# Autodesk Inventor assembly: full
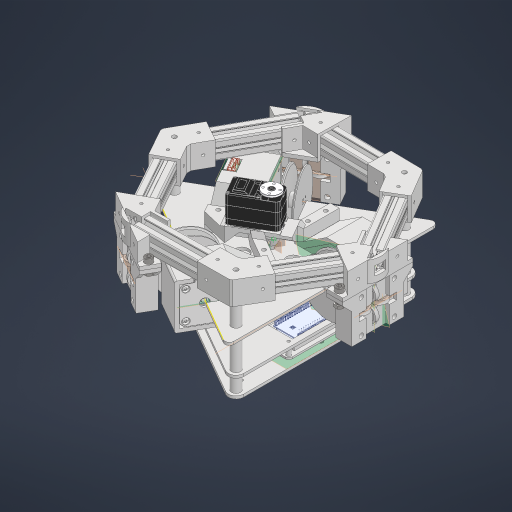
[picture p0: Inventor's stored thumbnail of the model, 512x512]
Saved by Autodesk Inventor 2024 (Build 280153000, 153)
## iProperties
Created: 2026-03-23
Part Number: full
Document SubType Name: Assembly
Designer: schar
Author: schar
## Documents named in this file (26)
- C:\Users\schar\Desktop\FloatingFace\models\full.iam
- C:\Users\schar\Desktop\FloatingFace\models\baseplate.ipt
- C:\Users\schar\Desktop\FloatingFace\models\spool.ipt
- C:\Users\schar\Desktop\FloatingFace\models\17HS4401S_Stepper_Motor\17HS4401S_Stepper_Motor.iam
- C:\Users\schar\Desktop\FloatingFace\models\esp32-s3-wroom-1-1.snapshot.2\ESP32-S3-WROOM-1\ESP32-S3-WROOM-1.iam
- C:\Users\schar\Desktop\FloatingFace\models\nema_brackets_and_lineguides.ipt
- C:\Users\schar\3D Objects\spacer_etage.ipt
- C:\Users\schar\3D Objects\second_etage.ipt
- C:\Users\schar\3D Objects\esp_spacer_fixed.ipt
- C:\Users\schar\Desktop\FloatingFace\models\esp_plate.ipt
- C:\Users\schar\Desktop\FloatingFace\models\guide.iam
- C:\Users\schar\Desktop\FloatingFace\models\2020_guide_adaptor.ipt
- C:\Users\schar\Desktop\FloatingFace\models\2020_top_guide_mnt.ipt
- C:\Users\schar\Desktop\FloatingFace\models\2020_nodes_conn.ipt
- C:\Users\schar\Desktop\FloatingFace\models\spacer_2020_node.ipt
- C:\Users\schar\Desktop\FloatingFace\models\2020_extrusion.ipt
- C:\Users\schar\Desktop\FloatingFace\models\ST3215 Servo.iam
- C:\Users\schar\Desktop\FloatingFace\models\servo_holder.ipt
- C:\Users\schar\Desktop\FloatingFace\models\servo_board_spacer.ipt
- C:\Users\schar\Desktop\FloatingFace\models\servo_rod_connector.ipt
- C:\Users\schar\Downloads\ROBOTIC_DOG_-STEP\drivers_pcb_v1.1.ipt
- C:\Users\schar\Desktop\FloatingFace\models\vertix_rod.ipt
- C:\Users\schar\Desktop\FloatingFace\models\multifunctional_lvl.ipt
- C:\Users\schar\Desktop\FloatingFace\models\multif_lvl_spacer.ipt
- C:\Users\schar\Documents\Inventor\Content Center Files\R2024\en-US\DIN 912\DIN 912 - M5 x 0,8 x 12 x 10.ipt
- C:\Users\schar\Documents\Inventor\Content Center Files\R2024\en-US\DIN 934\DIN 934 - M5 x 0,8.ipt
## Components (66 placed, 25 different names)
1. baseplate:1 — Mate:1, Mate:2, Mate:3, Mate:11, Mate:12, Flush:1, Mate:13, Mate:14, Mate:15, Flush:2, Flush:3, Flush:11, Flush:13, Mate:18, Mate:19, Mate:20, Mate:21, Flush:15, Mate:22, Mate:23, Angle:2, Angle:4, Flush:28, Mate:37, Mate:76, Mate:77, Mate:78
2. spool:1 — Mate:1, Mate:2, Mate:4, Mate:5
3. 17HS4401S_Stepper_Motor:1 [sub-assembly] — Mate:3, Mate:4, Mate:5
4. ESP32-S3-WROOM-1:1 [sub-assembly] — Mate:32, Flush:18, Flush:19
5. spool:2
6. 17HS4401S_Stepper_Motor:4 [sub-assembly] — Mate:14, Mate:15, Flush:2, Mate:16, Mate:17
7. spool:3 — Mate:11, Flush:4, Flush:20, Tangent:1, Tangent:2, Flush:24
8. 17HS4401S_Stepper_Motor:5 [sub-assembly] — Mate:12, Flush:1, Mate:13
9. nema_brackets_and_lineguides:1 — Flush:3, Flush:4, Flush:10, Angle:3, Angle:5
10. nema_brackets_and_lineguides:2 — Mate:16, Flush:11, Mate:17, Flush:12
11. spacer_etage:1 — Flush:13
12. spacer_etage:2 — Mate:18, Mate:19, Flush:14, Mate:31
13. spacer_etage:3 — Mate:20, Mate:21
14. second_etage:1 — Flush:14, Flush:16, Mate:25, Mate:26, Mate:27, Mate:28, Mate:29, Mate:30, Mate:31, Flush:35, Mate:80, Mate:81, Mate:82, Mate:83, Mate:84, Mate:85, Flush:41, Mate:86, Mate:87, Mate:88, Mate:89, Mate:90, Mate:91
15. nema_brackets_and_lineguides:3 — Flush:15, Mate:22, Mate:23, Mate:35, Flush:37
16. esp_spacer_fixed:1 — Flush:16, Flush:17
17. esp_spacer_fixed:2 — Mate:25, Mate:30
18. esp_spacer_fixed:3 — Mate:26, Mate:29
19. esp_spacer_fixed:4 — Mate:27, Mate:28
20. esp_plate:1 — Flush:17, Mate:32, Flush:18, Flush:19, Flush:39
21. drivers_pcb_v1.1:1
22. guide:2 [sub-assembly] — Mate:72, Mate:73, Mate:74
23. guide:3 [sub-assembly] — Mate:69, Mate:70, Mate:71
24. guide:1 [sub-assembly] — Mate:36, Flush:23, Flush:24, Flush:25
25. 2020_guide_adaptor:1 — Flush:25, Flush:26, Mate:104, Mate:106
26. 2020_top_guide_mnt:1 — Flush:26, Flush:29, Mate:55, Mate:56, Mate:57, Mate:95, Mate:96, Mate:101, Mate:102
27. 2020_nodes_conn:1 — Flush:27, Flush:30, Mate:38, Mate:39, Mate:40
28. spacer_2020_node:1 — Flush:27, Mate:37
29. 2020_extrusion:1 — Flush:29
30. 2020_extrusion:2 — Mate:38, Mate:39, Mate:40, Mate:41, Mate:42, Mate:43
31. spacer_2020_node:2 — Mate:50, Mate:51
32. 2020_nodes_conn:2 — Mate:47, Mate:48, Mate:49, Mate:50, Mate:51, Mate:52, Mate:53, Mate:54
33. 2020_top_guide_mnt:2 — Mate:41, Mate:42, Mate:43, Mate:44, Mate:45, Mate:46, Flush:33, Mate:68, Flush:34, Mate:72, Mate:97, Mate:98, Mate:99, Mate:100
34. 2020_extrusion:3 — Mate:44, Mate:45, Mate:46, Mate:47, Mate:48, Mate:49
35. 2020_extrusion:4 — Mate:55, Mate:56, Mate:57, Mate:58, Mate:59, Mate:60
36. 2020_extrusion:5 — Mate:52, Mate:53, Mate:54, Mate:65, Mate:66
37. 2020_extrusion:6 — Mate:61, Mate:62, Mate:63, Mate:64
38. 2020_top_guide_mnt:4 — Mate:64, Mate:65, Mate:66, Flush:31, Mate:67, Flush:32, Mate:71, Mate:92, Mate:93, Mate:94, Mate:107
39. 2020_nodes_conn:3 — Mate:58, Mate:59, Mate:60, Mate:61, Mate:62, Mate:63, Mate:75
40. 2020_guide_adaptor:2 — Flush:33, Mate:68, Flush:34, Mate:73, Mate:74, Mate:114
41. 2020_guide_adaptor:3 — Flush:31, Mate:67, Flush:32, Mate:69, Mate:70, Mate:109, Mate:111
42. spacer_2020_node:3 — Mate:75, Mate:76
43. ST3215 Servo:1 [sub-assembly] — Mate:77, Mate:78, Angle:5, Mate:79, Flush:36
44. servo_holder:1 — Mate:79
45. servo_board_spacer:1 — Flush:35
46. servo_board_spacer:2 — Mate:80, Mate:85
47. servo_board_spacer:3 — Mate:81, Mate:83
48. servo_board_spacer:4 — Mate:82, Mate:84
49. servo_rod_connector:1 — Flush:36, Flush:37, Flush:38
50. vertix_rod:1 — Flush:38
51. multifunctional_lvl:1 — Flush:40, Mate:90, Mate:91
52. multif_lvl_spacer:1 — Flush:41
53. multif_lvl_spacer:2 — Mate:86, Mate:89
54. multif_lvl_spacer:3 — Mate:87, Mate:88
55. DIN 912 - replaced by DIN EN ISO 4762 M5 x 12:1 — Mate:92, Mate:93, Mate:110
56. DIN 912 - replaced by DIN EN ISO 4762 M5 x 12:2 — Mate:94, Mate:107, Mate:108
57. DIN 912 - replaced by DIN EN ISO 4762 M5 x 12:3 — Mate:95, Mate:102, Mate:103
58. DIN 912 - replaced by DIN EN ISO 4762 M5 x 12:4 — Mate:96, Mate:101, Mate:105
59. DIN 912 - replaced by DIN EN ISO 4762 M5 x 12:5 — Mate:97, Mate:100, Mate:112
60. DIN 912 - replaced by DIN EN ISO 4762 M5 x 12:6 — Mate:98, Mate:99, Mate:113
61. DIN 934 - replaced by DIN EN 24032/28673/28674 M5:1 — Mate:103, Mate:104
62. DIN 934 - replaced by DIN EN 24032/28673/28674 M5:2 — Mate:105, Mate:106
63. DIN 934 - replaced by DIN EN 24032/28673/28674 M5:3 — Mate:108, Mate:109
64. DIN 934 - replaced by DIN EN 24032/28673/28674 M5:4 — Mate:110, Mate:111
65. DIN 934 - replaced by DIN EN 24032/28673/28674 M5:5 — Mate:112, Mate:114
66. DIN 934 - replaced by DIN EN 24032/28673/28674 M5:6 — Mate:113
## Relationships (154: Mate 112, Flush 35, Angle 5, Tangent 2)
- Mate:1: baseplate:1 ↔ spool:1
- Mate:2: baseplate:1 ↔ spool:1
- Mate:3: baseplate:1 ↔ 17HS4401S_Stepper_Motor:1
- Mate:4: spool:1 ↔ 17HS4401S_Stepper_Motor:1
- Mate:5: spool:1 ↔ 17HS4401S_Stepper_Motor:1
- [Mate]: spool:2 ↔ 17HS4401S_Stepper_Motor:4
- [Mate]: spool:2 ↔ 17HS4401S_Stepper_Motor:4
- [Mate]: spool:3 ↔ 17HS4401S_Stepper_Motor:5
- [Mate]: spool:3 ↔ 17HS4401S_Stepper_Motor:5
- Mate:11: baseplate:1 ↔ spool:3
- Mate:12: baseplate:1 ↔ 17HS4401S_Stepper_Motor:5
- Flush:1: baseplate:1 ↔ 17HS4401S_Stepper_Motor:5
- Mate:13: baseplate:1 ↔ 17HS4401S_Stepper_Motor:5
- Mate:14: baseplate:1 ↔ 17HS4401S_Stepper_Motor:4
- Mate:15: baseplate:1 ↔ 17HS4401S_Stepper_Motor:4
- Flush:2: baseplate:1 ↔ 17HS4401S_Stepper_Motor:4
- Flush:3: baseplate:1 ↔ nema_brackets_and_lineguides:1
- Flush:4 (2 mm): spool:3 ↔ nema_brackets_and_lineguides:1
- Flush:10: nema_brackets_and_lineguides:1
- Mate:16: 17HS4401S_Stepper_Motor:4 ↔ nema_brackets_and_lineguides:2
- Flush:11: baseplate:1 ↔ nema_brackets_and_lineguides:2
- Mate:17: 17HS4401S_Stepper_Motor:4 ↔ nema_brackets_and_lineguides:2
- Flush:12: nema_brackets_and_lineguides:2
- Flush:13: baseplate:1 ↔ spacer_etage:1
- Mate:18: baseplate:1 ↔ spacer_etage:2
- Mate:19: baseplate:1 ↔ spacer_etage:2
- Mate:20: baseplate:1 ↔ spacer_etage:3
- Mate:21: baseplate:1 ↔ spacer_etage:3
- Flush:14: spacer_etage:2 ↔ second_etage:1
- Flush:15: baseplate:1 ↔ nema_brackets_and_lineguides:3
- Mate:22: baseplate:1 ↔ nema_brackets_and_lineguides:3
- Mate:23: baseplate:1 ↔ nema_brackets_and_lineguides:3
- Flush:16: second_etage:1 ↔ esp_spacer_fixed:1
- Mate:25: second_etage:1 ↔ esp_spacer_fixed:2
- Mate:26: second_etage:1 ↔ esp_spacer_fixed:3
- Mate:27: second_etage:1 ↔ esp_spacer_fixed:4
- Mate:28: second_etage:1 ↔ esp_spacer_fixed:4
- Mate:29: second_etage:1 ↔ esp_spacer_fixed:3
- Mate:30: second_etage:1 ↔ esp_spacer_fixed:2
- Mate:31: spacer_etage:2 ↔ second_etage:1
- Flush:17: esp_spacer_fixed:1 ↔ esp_plate:1
- Mate:32: ESP32-S3-WROOM-1:1 ↔ esp_plate:1
- Flush:18: ESP32-S3-WROOM-1:1 ↔ esp_plate:1
- Flush:19: ESP32-S3-WROOM-1:1 ↔ esp_plate:1
- [Mate]: second_etage:1 ↔ drivers_pcb_v1.1:1
- [Mate]: second_etage:1 ↔ drivers_pcb_v1.1:1
- [Angle] (0 deg): second_etage:1 ↔ drivers_pcb_v1.1:1
- Mate:35: nema_brackets_and_lineguides:3
- Angle:2 (90 deg): baseplate:1
- Flush:20: spool:3
- Angle:3 (0 deg): nema_brackets_and_lineguides:1
- Tangent:1: spool:3
- Flush:21 (5 mm)
- Mate:36: guide:1
- Angle:4 (0 deg): baseplate:1
- Tangent:2: spool:3
- Flush:23: guide:1
- Flush:24: spool:3 ↔ guide:1
- Flush:25: guide:1 ↔ 2020_guide_adaptor:1
- Flush:26: 2020_guide_adaptor:1 ↔ 2020_top_guide_mnt:1
- Flush:27: 2020_nodes_conn:1 ↔ spacer_2020_node:1
- Flush:28: baseplate:1
- Mate:37: baseplate:1 ↔ spacer_2020_node:1
- Flush:29: 2020_top_guide_mnt:1 ↔ 2020_extrusion:1
- Flush:30: 2020_nodes_conn:1
- Mate:38: 2020_nodes_conn:1 ↔ 2020_extrusion:2
- Mate:39: 2020_nodes_conn:1 ↔ 2020_extrusion:2
- Mate:40: 2020_nodes_conn:1 ↔ 2020_extrusion:2
- Mate:41: 2020_extrusion:2 ↔ 2020_top_guide_mnt:2
- Mate:42: 2020_extrusion:2 ↔ 2020_top_guide_mnt:2
- Mate:43: 2020_extrusion:2 ↔ 2020_top_guide_mnt:2
- Mate:44: 2020_top_guide_mnt:2 ↔ 2020_extrusion:3
- Mate:45: 2020_top_guide_mnt:2 ↔ 2020_extrusion:3
- Mate:46: 2020_top_guide_mnt:2 ↔ 2020_extrusion:3
- Mate:47: 2020_nodes_conn:2 ↔ 2020_extrusion:3
- Mate:48: 2020_nodes_conn:2 ↔ 2020_extrusion:3
- Mate:49: 2020_nodes_conn:2 ↔ 2020_extrusion:3
- Mate:50: spacer_2020_node:2 ↔ 2020_nodes_conn:2
- Mate:51: spacer_2020_node:2 ↔ 2020_nodes_conn:2
- Mate:52: 2020_nodes_conn:2 ↔ 2020_extrusion:5
- Mate:53: 2020_nodes_conn:2 ↔ 2020_extrusion:5
- Mate:54: 2020_nodes_conn:2 ↔ 2020_extrusion:5
- Mate:55: 2020_top_guide_mnt:1 ↔ 2020_extrusion:4
- Mate:56: 2020_top_guide_mnt:1 ↔ 2020_extrusion:4
- Mate:57: 2020_top_guide_mnt:1 ↔ 2020_extrusion:4
- Mate:58: 2020_extrusion:4 ↔ 2020_nodes_conn:3
- Mate:59: 2020_extrusion:4 ↔ 2020_nodes_conn:3
- Mate:60: 2020_extrusion:4 ↔ 2020_nodes_conn:3
- Mate:61: 2020_extrusion:6 ↔ 2020_nodes_conn:3
- Mate:62: 2020_extrusion:6 ↔ 2020_nodes_conn:3
- Mate:63: 2020_extrusion:6 ↔ 2020_nodes_conn:3
- Mate:64: 2020_extrusion:6 ↔ 2020_top_guide_mnt:4
- Mate:65: 2020_extrusion:5 ↔ 2020_top_guide_mnt:4
- Mate:66: 2020_extrusion:5 ↔ 2020_top_guide_mnt:4
- Flush:31: 2020_top_guide_mnt:4 ↔ 2020_guide_adaptor:3
- Mate:67: 2020_top_guide_mnt:4 ↔ 2020_guide_adaptor:3
- Flush:32: 2020_top_guide_mnt:4 ↔ 2020_guide_adaptor:3
- Flush:33: 2020_top_guide_mnt:2 ↔ 2020_guide_adaptor:2
- Mate:68: 2020_top_guide_mnt:2 ↔ 2020_guide_adaptor:2
- Flush:34: 2020_top_guide_mnt:2 ↔ 2020_guide_adaptor:2
- Mate:69: guide:3 ↔ 2020_guide_adaptor:3
- Mate:70: guide:3 ↔ 2020_guide_adaptor:3
- Mate:71: guide:3 ↔ 2020_top_guide_mnt:4
- Mate:72: guide:2 ↔ 2020_top_guide_mnt:2
- Mate:73: guide:2 ↔ 2020_guide_adaptor:2
- Mate:74: guide:2 ↔ 2020_guide_adaptor:2
- Mate:75: 2020_nodes_conn:3 ↔ spacer_2020_node:3
- Mate:76: baseplate:1 ↔ spacer_2020_node:3
- Mate:77: baseplate:1 ↔ ST3215 Servo:1
- Mate:78 (20 mm): baseplate:1 ↔ ST3215 Servo:1
- Angle:5 (0 deg): nema_brackets_and_lineguides:1 ↔ ST3215 Servo:1
- Mate:79: ST3215 Servo:1 ↔ servo_holder:1
- Flush:35: second_etage:1 ↔ servo_board_spacer:1
- Mate:80: second_etage:1 ↔ servo_board_spacer:2
- Mate:81: second_etage:1 ↔ servo_board_spacer:3
- Mate:82: second_etage:1 ↔ servo_board_spacer:4
- Mate:83: second_etage:1 ↔ servo_board_spacer:3
- Mate:84: second_etage:1 ↔ servo_board_spacer:4
- Mate:85: second_etage:1 ↔ servo_board_spacer:2
- Flush:36: ST3215 Servo:1 ↔ servo_rod_connector:1
- Flush:37: nema_brackets_and_lineguides:3 ↔ servo_rod_connector:1
- Flush:38: servo_rod_connector:1 ↔ vertix_rod:1
- Flush:39 (5 mm): esp_plate:1
- Flush:40: multifunctional_lvl:1
- Flush:41: second_etage:1 ↔ multif_lvl_spacer:1
- Mate:86: second_etage:1 ↔ multif_lvl_spacer:2
- Mate:87: second_etage:1 ↔ multif_lvl_spacer:3
- Mate:88: second_etage:1 ↔ multif_lvl_spacer:3
- Mate:89: second_etage:1 ↔ multif_lvl_spacer:2
- Mate:90: second_etage:1 ↔ multifunctional_lvl:1
- Mate:91: second_etage:1 ↔ multifunctional_lvl:1
- Mate:92: 2020_top_guide_mnt:4 ↔ DIN 912 - replaced by DIN EN ISO 4762 M5 x 12:1
- Mate:93: 2020_top_guide_mnt:4 ↔ DIN 912 - replaced by DIN EN ISO 4762 M5 x 12:1
- Mate:94: 2020_top_guide_mnt:4 ↔ DIN 912 - replaced by DIN EN ISO 4762 M5 x 12:2
- Mate:95: 2020_top_guide_mnt:1 ↔ DIN 912 - replaced by DIN EN ISO 4762 M5 x 12:3
- Mate:96: 2020_top_guide_mnt:1 ↔ DIN 912 - replaced by DIN EN ISO 4762 M5 x 12:4
- Mate:97: 2020_top_guide_mnt:2 ↔ DIN 912 - replaced by DIN EN ISO 4762 M5 x 12:5
- Mate:98: 2020_top_guide_mnt:2 ↔ DIN 912 - replaced by DIN EN ISO 4762 M5 x 12:6
- Mate:99: 2020_top_guide_mnt:2 ↔ DIN 912 - replaced by DIN EN ISO 4762 M5 x 12:6
- Mate:100: 2020_top_guide_mnt:2 ↔ DIN 912 - replaced by DIN EN ISO 4762 M5 x 12:5
- Mate:101: 2020_top_guide_mnt:1 ↔ DIN 912 - replaced by DIN EN ISO 4762 M5 x 12:4
- Mate:102: 2020_top_guide_mnt:1 ↔ DIN 912 - replaced by DIN EN ISO 4762 M5 x 12:3
- Mate:103: DIN 912 - replaced by DIN EN ISO 4762 M5 x 12:3 ↔ DIN 934 - replaced by DIN EN 24032/28673/28674 M5:1
- Mate:104: 2020_guide_adaptor:1 ↔ DIN 934 - replaced by DIN EN 24032/28673/28674 M5:1
- Mate:105: DIN 912 - replaced by DIN EN ISO 4762 M5 x 12:4 ↔ DIN 934 - replaced by DIN EN 24032/28673/28674 M5:2
- Mate:106: 2020_guide_adaptor:1 ↔ DIN 934 - replaced by DIN EN 24032/28673/28674 M5:2
- Mate:107: 2020_top_guide_mnt:4 ↔ DIN 912 - replaced by DIN EN ISO 4762 M5 x 12:2
- Mate:108: DIN 912 - replaced by DIN EN ISO 4762 M5 x 12:2 ↔ DIN 934 - replaced by DIN EN 24032/28673/28674 M5:3
- Mate:109: 2020_guide_adaptor:3 ↔ DIN 934 - replaced by DIN EN 24032/28673/28674 M5:3
- Mate:110: DIN 912 - replaced by DIN EN ISO 4762 M5 x 12:1 ↔ DIN 934 - replaced by DIN EN 24032/28673/28674 M5:4
- Mate:111: 2020_guide_adaptor:3 ↔ DIN 934 - replaced by DIN EN 24032/28673/28674 M5:4
- Mate:112: DIN 912 - replaced by DIN EN ISO 4762 M5 x 12:5 ↔ DIN 934 - replaced by DIN EN 24032/28673/28674 M5:5
- Mate:113: DIN 912 - replaced by DIN EN ISO 4762 M5 x 12:6 ↔ DIN 934 - replaced by DIN EN 24032/28673/28674 M5:6
- Mate:114: 2020_guide_adaptor:2 ↔ DIN 934 - replaced by DIN EN 24032/28673/28674 M5:5
## Named parameters: d8_d5 = 0 mm, d9_d6 = 0 mm, d10_d5 = 0 mm, d11_d6 = 0 mm
